# Autodesk Inventor assembly: Assemblywithlid
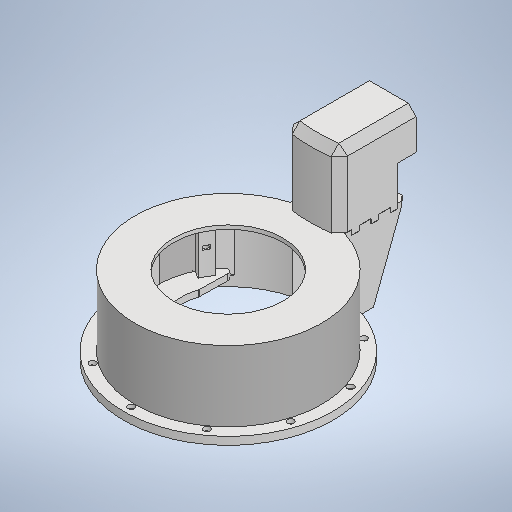
[picture p0: Inventor's stored thumbnail of the model, 512x512]
Saved by Autodesk Inventor 2025.2 (Build 292293000, 293)
## iProperties
Created: 2025-08-14
Part Number: Assemblywithlid
Document SubType Name: Assembly
Designer: mateo
Author: mateo
## Documents named in this file (4)
- C:\GitHub\In-situ-monitoring-of-powder-bed-fusion-additive-manufacturing\system_development\Adamant\v0.2\hardware_development\Assemblywithlid.iam
- C:\GitHub\In-situ-monitoring-of-powder-bed-fusion-additive-manufacturing\system_development\Adamant\v0.2\hardware_development\Cover parts\Cylinder Segment Holder.ipt
- C:\GitHub\In-situ-monitoring-of-powder-bed-fusion-additive-manufacturing\system_development\Adamant\v0.2\hardware_development\Cover parts\Cylinder Slidey Bit Housing Camera v0.2.1.ipt
- C:\GitHub\In-situ-monitoring-of-powder-bed-fusion-additive-manufacturing\system_development\Adamant\v0.2\hardware_development\Cover parts\thermal camera lid.ipt
## Components (3 placed, 3 different names)
1. Cylinder Segment Holder:1 — Insert:1
2. Cylinder Slidey Bit Housing Camera v0.2.1:1 — Insert:1, Mate:1, Mate:2, Mate:3
3. thermal camera lid:1 — Mate:1, Mate:2, Mate:3
## Relationships (4: Mate 3, Insert 1)
- Insert:1: Cylinder Segment Holder:1 ↔ Cylinder Slidey Bit Housing Camera v0.2.1:1
- Mate:1: Cylinder Slidey Bit Housing Camera v0.2.1:1 ↔ thermal camera lid:1
- Mate:2: Cylinder Slidey Bit Housing Camera v0.2.1:1 ↔ thermal camera lid:1
- Mate:3: Cylinder Slidey Bit Housing Camera v0.2.1:1 ↔ thermal camera lid:1
